# Autodesk Inventor assembly: Montagem6
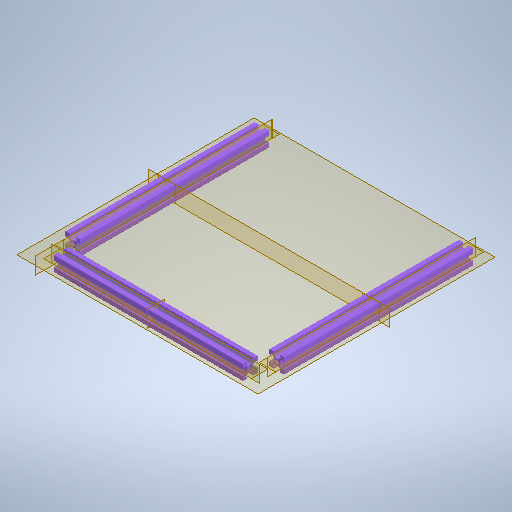
[picture p0: Inventor's stored thumbnail of the model, 512x512]
Saved by Autodesk Inventor 2025.2 (Build 292293000, 293)
## iProperties
Created: 2025-03-28
Part Number: Montagem6
Document SubType Name: Assembly
Designer: Formação
Author: Formação
## Documents named in this file (2)
- C:\Users\Formação\Documents\Inventor\Sessão_25_03_25\Montagem6.iam
- C:\Users\Formação\Documents\Inventor\Sessão_25_03_25\Peça2.ipt
## Components (3 placed, 1 different names)
1. Peça2:1 — Alinhado:1, Coincidente:1, Coincidente:2, Coincidente:3, Coincidente:4, Coincidente:5, Coincidente:6, Coincidente:7, Coincidente:8, Coincidente:10, Coincidente:11
2. Peça2:2 — Alinhado:3, Alinhado:4, Coincidente:9
3. Peça2:3 — Coincidente:3, Coincidente:4, Coincidente:5, Alinhado:2, Coincidente:6, Coincidente:7, Coincidente:8, Coincidente:9, Coincidente:10, Coincidente:11
## Relationships (15: Mate 11, Flush 4)
- Alinhado:1 [Flush]: Peça2:1
- Coincidente:1 [Mate]: Peça2:1
- Coincidente:2 [Mate]: Peça2:1
- Coincidente:3 [Mate]: Peça2:1 ↔ Peça2:3
- Coincidente:4 [Mate]: Peça2:1 ↔ Peça2:3
- Coincidente:5 [Mate]: Peça2:1 ↔ Peça2:3
- Alinhado:2 [Flush]: Peça2:3
- Coincidente:6 [Mate]: Peça2:1 ↔ Peça2:3
- Coincidente:7 [Mate]: Peça2:1 ↔ Peça2:3
- Coincidente:8 [Mate]: Peça2:1 ↔ Peça2:3
- Alinhado:3 [Flush]: Peça2:2
- Alinhado:4 [Flush]: Peça2:2
- Coincidente:9 [Mate]: Peça2:2 ↔ Peça2:3
- Coincidente:10 [Mate]: Peça2:1 ↔ Peça2:3
- Coincidente:11 [Mate]: Peça2:1 ↔ Peça2:3
